# Autodesk Inventor assembly: FelAlvaz
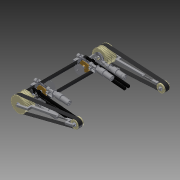
[picture p0: Inventor's stored thumbnail of the model, 180x180]
Saved by Autodesk Inventor 2015 (Build 190159000, 159)
## iProperties
Created: 2015-02-23
Part Number: FelAlvaz
Document SubType Name: Assembly
Designer: laca
Author: laca
## Documents named in this file (10)
- C:\Users\laca\Desktop\iRoobo2014Ver3\FelAlvaz.iam
- C:\Users\laca\Desktop\iRoobo2014Ver3\CsapágyHáz.ipt
- C:\Users\laca\Desktop\iRoobo2014Ver3\EgyvégenMartSzelvény.ipt
- C:\Users\laca\Desktop\iRoobo2014Ver3\KétvégenMartSzelvény.ipt
- C:\Users\laca\Desktop\iRoobo2014Ver3\6001 BEARING.iam
- C:\Users\laca\Desktop\iRoobo2014Ver3\ProvedoSenzor.iam
- C:\Users\laca\Desktop\iRoobo2014Ver3\Talp.iam
- C:\Users\laca\Desktop\iRoobo2014Ver3\KozepsoOsszekotok.ipt
- C:\Users\laca\Desktop\iRoobo2014Ver3\SzéleségiSzelvény.ipt
- C:\Users\laca\Desktop\iRoobo2014Ver3\ProvedoSenzor Tukrozot.iam
## Components (21 placed, 9 different names)
1. CsapágyHáz:1
2. EgyvégenMartSzelvény:1
3. KétvégenMartSzelvény:1
4. EgyvégenMartSzelvény:3 — Rigid:11
5. KétvégenMartSzelvény:2 — Flush:3
6. 6001 BEARING:2 [sub-assembly]
7. 6001 BEARING:4 [sub-assembly] — Insert:7
8. ProvedoSenzor:1 [sub-assembly]
9. ProvedoSenzor Tukrozot:1 [sub-assembly] — Insert:12, Flush:6
10. ProvedoSenzor:2 [sub-assembly]
11. Talp:1 [sub-assembly] — Insert:7, Flush:3, Flush:8, Flush:9, Flush:12
12. Talp:2 [sub-assembly] — Flush:5, Flush:10, Flush:11, Mate:11, Mate:16
13. KozepsoOsszekotok:1 — Flush:7, Mate:1, Mate:2, Mate:11, Mate:12, Mate:13, Flush:12
14. SzéleségiSzelvény:1 — Rigid:11, Rigid:16, Mate:2, Flush:8, Flush:9, Flush:10, Flush:11
15. CsapágyHáz:2 — Insert:12
16. EgyvégenMartSzelvény:4
17. KétvégenMartSzelvény:3 — Flush:7, Mate:1
18. EgyvégenMartSzelvény:5 — Rigid:16
19. KétvégenMartSzelvény:4 — Flush:5, Flush:6
20. 6001 BEARING:5 [sub-assembly]
21. 6001 BEARING:6 [sub-assembly]
## Relationships (39: Flush 11, WeldJoint 10, Insert 9, Mate 9)
- [WeldJoint]: CsapágyHáz:1 ↔ KétvégenMartSzelvény:2
- [WeldJoint]: CsapágyHáz:1 ↔ KétvégenMartSzelvény:1
- [WeldJoint]: CsapágyHáz:1 ↔ EgyvégenMartSzelvény:1
- [WeldJoint]: CsapágyHáz:1 ↔ EgyvégenMartSzelvény:3
- [Insert]: CsapágyHáz:1 ↔ 6001 BEARING:2
- [Insert]: CsapágyHáz:1 ↔ 6001 BEARING:4
- [Insert]: CsapágyHáz:1 ↔ ProvedoSenzor:1
- [Flush]: KétvégenMartSzelvény:2 ↔ ProvedoSenzor:1
- Insert:7: 6001 BEARING:4 ↔ Talp:1
- Flush:3: KétvégenMartSzelvény:2 ↔ Talp:1
- Rigid:11 [WeldJoint]: EgyvégenMartSzelvény:3 ↔ SzéleségiSzelvény:1
- [WeldJoint]: CsapágyHáz:2 ↔ KétvégenMartSzelvény:4
- [WeldJoint]: CsapágyHáz:2 ↔ KétvégenMartSzelvény:3
- [WeldJoint]: CsapágyHáz:2 ↔ EgyvégenMartSzelvény:4
- [WeldJoint]: CsapágyHáz:2 ↔ EgyvégenMartSzelvény:5
- [Insert]: CsapágyHáz:2 ↔ 6001 BEARING:5
- [Insert]: CsapágyHáz:2 ↔ 6001 BEARING:6
- [Insert]: ProvedoSenzor:2 ↔ CsapágyHáz:2
- [Flush]: ProvedoSenzor:2 ↔ KétvégenMartSzelvény:4
- [Insert]: Talp:2 ↔ 6001 BEARING:6
- Flush:5: Talp:2 ↔ KétvégenMartSzelvény:4
- Rigid:16 [WeldJoint]: SzéleségiSzelvény:1 ↔ EgyvégenMartSzelvény:5
- Insert:12: ProvedoSenzor Tukrozot:1 ↔ CsapágyHáz:2
- Flush:6: ProvedoSenzor Tukrozot:1 ↔ KétvégenMartSzelvény:4
- Flush:7: KozepsoOsszekotok:1 ↔ KétvégenMartSzelvény:3
- Mate:1: KozepsoOsszekotok:1 ↔ KétvégenMartSzelvény:3
- Mate:2 (100 mm): KozepsoOsszekotok:1 ↔ SzéleségiSzelvény:1
- Flush:8 (-2 mm): Talp:1 ↔ SzéleségiSzelvény:1
- Flush:9: Talp:1 ↔ SzéleségiSzelvény:1
- Flush:10: Talp:2 ↔ SzéleségiSzelvény:1
- Flush:11 (-2 mm): Talp:2 ↔ SzéleségiSzelvény:1
- Mate:11: Talp:2 ↔ KozepsoOsszekotok:1
- Mate:12: KozepsoOsszekotok:1
- Mate:13: KozepsoOsszekotok:1
- Mate:14
- Mate:15
- Mate:16: Talp:2
- Mate:17
- Flush:12: Talp:1 ↔ KozepsoOsszekotok:1
## Named parameters: d14_d18 = 0 mm, d16_d20 = 0 mm, d54_d22 = 0 mm, d55_d23 = 30 mm, d56_d24 = -30 mm, d57_d8 = 0 mm, d58_d9 = 0 mm, d59_d14_d18 = 0 mm, d60_d16_d20 = 0 mm, d61_d21 = 0 mm, d62_d0 = 0 mm, d63_d1 = -70.13484 deg, d64_d2 = 0 mm, d65_d25 = 0 mm, d66_d30 = 0 mm, d67_d31 = 254 mm, d68_d32 = -254 mm
